# Autodesk Inventor assembly: UpperArm_diagonal
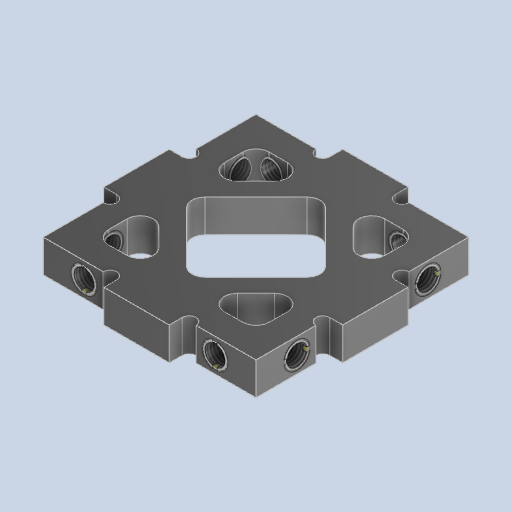
[picture p0: Inventor's stored thumbnail of the model, 512x512]
Saved by Autodesk Inventor 2022.5 (Build 265521000, 521)
## iProperties
Created: 2023-06-02
Part Number: UpperArm_diagonal
Document SubType Name: Assembly
Designer: Masato Kubotera
Author: Masato Kubotera
## Documents named in this file (3)
- C:\Users\Masato\Documents\Inventor\SUSTAINA-OP\ModelingFiles\UpperBody\Arm\UpperArm_diagonal.iam
- C:\Users\Masato\Documents\Inventor\SUSTAINA-OP\ModelingFiles\UpperBody\Arm\UpperArm_diagonal.ipt
- C:\Users\Masato\Documents\Inventor\SUSTAINA-OP\ModelingFiles\COTS\InsertNut\IRU-304S.ipt
## Components (9 placed, 2 different names)
1. UpperArm_diagonal:1 — Insert:1, Insert:2, Insert:3, Insert:4, Insert:5, Insert:6, Insert:7, Insert:8
2. IRU-304S:1 — Insert:1
3. IRU-304S:2 — Insert:2
4. IRU-304S:3 — Insert:3
5. IRU-304S:4 — Insert:4
6. IRU-304S:5 — Insert:5
7. IRU-304S:6 — Insert:6
8. IRU-304S:7 — Insert:7
9. IRU-304S:8 — Insert:8
## Relationships (8: Insert 8)
- Insert:1: UpperArm_diagonal:1 ↔ IRU-304S:1
- Insert:2: UpperArm_diagonal:1 ↔ IRU-304S:2
- Insert:3: UpperArm_diagonal:1 ↔ IRU-304S:3
- Insert:4: UpperArm_diagonal:1 ↔ IRU-304S:4
- Insert:5: UpperArm_diagonal:1 ↔ IRU-304S:5
- Insert:6: UpperArm_diagonal:1 ↔ IRU-304S:6
- Insert:7: UpperArm_diagonal:1 ↔ IRU-304S:7
- Insert:8: UpperArm_diagonal:1 ↔ IRU-304S:8
